# Autodesk Inventor assembly: Screw_Joint_36T
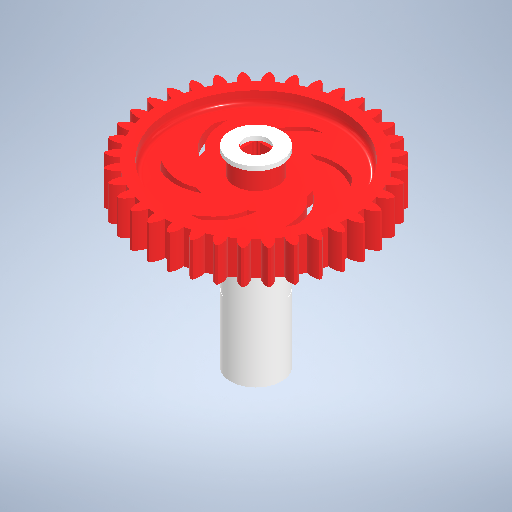
[picture p0: Inventor's stored thumbnail of the model, 512x512]
Saved by Autodesk Inventor 2025 (Build 290162000, 162)
## iProperties
Created: 2024-12-08
Part Number: Screw_Joint_36T
Document SubType Name: Assembly
Designer: Aditya Koduri
Author: Aditya Koduri
## Documents named in this file (6)
- C:\Users\mzart\Downloads\Full_Cad_Model\Screw_Joint_36T.iam
- C:\Users\mzart\Downloads\VEX-CAD-Inventor-main\VEX-CAD-Inventor-main\Motion\Gears\LS 36T Gear.ipt
- C:\Users\mzart\Downloads\VEX-CAD-Inventor-main\VEX-CAD-Inventor-main\Motion\Spacers\Washer Teflon\TWasher .375 OD x .03125.ipt
- C:\Users\mzart\Downloads\VEX-CAD-Inventor-main\VEX-CAD-Inventor-main\Motion\Spacers\Spacer Nylon .313 OD\NSpacer .313 OD x .500.ipt
- C:\Users\mzart\Downloads\VEX-CAD-Inventor-main\VEX-CAD-Inventor-main\Motion\Spacers\Washer Teflon.ipt
- C:\Users\mzart\Downloads\VEX-CAD-Inventor-main\VEX-CAD-Inventor-main\Motion\Spacers\Spacer Nylon .313 OD.ipt
## Components (4 placed, 3 different names)
1. LS 36T Gear:1 — Insert:2
2. TWasher .375 OD x .03125:1
3. NSpacer .313 OD x .500:1 — Insert:2, Insert:3
4. NSpacer .313 OD x .500:2 — Insert:3
## Relationships (3: Insert 3)
- [Insert]: LS 36T Gear:1 ↔ TWasher .375 OD x .03125:1
- Insert:2: LS 36T Gear:1 ↔ NSpacer .313 OD x .500:1
- Insert:3: NSpacer .313 OD x .500:1 ↔ NSpacer .313 OD x .500:2
## Named parameters: d119_d118 = 0 mm
